# Autodesk Inventor assembly: Assembly_v2
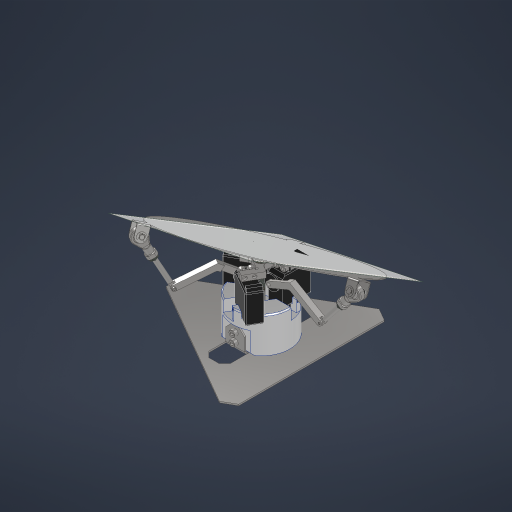
[picture p0: Inventor's stored thumbnail of the model, 512x512]
Saved by Autodesk Inventor 2023 (Build 270158000, 158)
## iProperties
Created: 2023-02-25
Part Number: Assembly_v2
Document SubType Name: Assembly
Designer: roota
Mass: 2527.07 g
Surface Area: 3464.46 cm^2
Volume: 460 cm^3
Density: 5.49363 g/cm^3
Author: roota
## Documents named in this file (20)
- D:\GitHub\NTUST-Mechanical-Design\Ball stabilization mechanism\3D CAD files\Mechanical Part CAD files\Assemblies\Assembly_v2.iam
- D:\GitHub\NTUST-Mechanical-Design\Ball stabilization mechanism\3D CAD files\Mechanical Part CAD files\Static Mechanisms\BalancePlate.ipt
- D:\GitHub\NTUST-Mechanical-Design\Ball stabilization mechanism\3D CAD files\Mechanical Part CAD files\Static Mechanisms\BasePlate.ipt
- D:\GitHub\NTUST-Mechanical-Design\Ball stabilization mechanism\3D CAD files\Mechanical Part CAD files\Static Mechanisms\BaseSupport.ipt
- D:\GitHub\NTUST-Mechanical-Design\Ball stabilization mechanism\3D CAD files\Mechanical Part CAD files\Static Mechanisms\ServoCap.ipt
- D:\GitHub\NTUST-Mechanical-Design\Ball stabilization mechanism\3D CAD files\Electrical Hardware CAD files\SERVO\LDX-335MG_Servo_15kg_cm.ipt
- C:\Users\roota\Documents\Inventor\Content Center Files\R2023\en-US\ISO 10642(1)\ISO 10642 - M8 x  60.ipt
- C:\Users\roota\Documents\Inventor\Content Center Files\R2023\en-US\ISO 4762(2)\ISO 4762 - M5 x 8ISO.ipt
- C:\Users\roota\Documents\Inventor\Content Center Files\R2023\en-US\ISO 4026\ISO 4026 - M3 x 6 - ISO.ipt
- D:\GitHub\NTUST-Mechanical-Design\Ball stabilization mechanism\3D CAD files\Mechanical Part CAD files\Hardware Parts\5mm Bushing.ipt
- D:\GitHub\NTUST-Mechanical-Design\Ball stabilization mechanism\3D CAD files\Mechanical Part CAD files\Hardware Parts\M6x1_THREADED_ROD.ipt
- C:\Users\roota\Documents\Inventor\Content Center Files\R2023\en-US\ISO 4762(2)\ISO 4762 - M2.5 x 8ISO.ipt
- D:\GitHub\NTUST-Mechanical-Design\Ball stabilization mechanism\3D CAD files\Mechanical Part CAD files\Hardware Parts\SELF-LUBRIFICATING ROD END\End_6mm.ipt
- D:\GitHub\NTUST-Mechanical-Design\Ball stabilization mechanism\3D CAD files\Mechanical Part CAD files\Hardware Parts\SELF-LUBRIFICATING ROD END\Ball_6mm.ipt
- D:\GitHub\NTUST-Mechanical-Design\Ball stabilization mechanism\3D CAD files\Mechanical Part CAD files\Static Mechanisms\4mm spacer.ipt
- D:\GitHub\NTUST-Mechanical-Design\Ball stabilization mechanism\3D CAD files\Mechanical Part CAD files\Static Mechanisms\rod pin.ipt
- C:\Users\roota\Documents\Inventor\Content Center Files\R2023\en-US\JIS B 2804 E\_JIS B 2804 E - 5 - 6.ipt
- C:\Users\roota\Documents\Inventor\Content Center Files\R2023\en-US\ISO 4036(2)\ISO 4036 - M6(2).ipt
- D:\GitHub\NTUST-Mechanical-Design\Ball stabilization mechanism\3D CAD files\Mechanical Part CAD files\Hardware Parts\12_1_INCH_TOUCHSCREEN\12inch Touchscreen.ipt
- D:\GitHub\NTUST-Mechanical-Design\Ball stabilization mechanism\3D CAD files\Mechanical Part CAD files\Dynamic Mechanisms\Servo_Strut_v2.ipt
## Components (58 placed, 19 different names)
1. BalancePlate:1 — Mate:19, Mate:20, Mate:21, Mate:22, Mate:23, Mate:24, Mate:26, Mate:28, Mate:30, Mate:31, Flush:1, Flush:2, Mate:44
2. BasePlate:1 — Mate:1, Mate:2, Mate:3, Insert:13, Insert:14, Insert:15, Insert:16, Angle:4, Angle:5
3. BaseSupport:1 — Mate:1, Mate:2, Mate:3, Mate:4, Mate:5, Mate:6, Mate:7, Mate:8, Mate:9, Mate:10, Mate:11, Mate:12, Mate:17, Mate:18, Insert:17, Mate:44
4. ServoCap:1 — Mate:13, Mate:14, Mate:15, Mate:16
5. LDX-335MG_Servo_15kg_cm:1 — Mate:4, Mate:7, Mate:10, Insert:5, Insert:8, Insert:49
6. LDX-335MG_Servo_15kg_cm:2 — Mate:5, Mate:8, Mate:11, Insert:9, Insert:12, Insert:50
7. LDX-335MG_Servo_15kg_cm:3 — Mate:6, Mate:9, Mate:12, Mate:13, Mate:14, Mate:15, Insert:1, Insert:4, Insert:48
8. ISO 10642 M8x60:1 — Mate:16
9. ISO 4762 M5 x 8:1 — Insert:1
10. ISO 4762 M5 x 8:4 — Insert:4
11. ISO 4762 M5 x 8:5 — Insert:5
12. ISO 4762 M5 x 8:8 — Insert:8
13. ISO 4762 M5 x 8:9 — Insert:9
14. ISO 4762 M5 x 8:12 — Insert:12
15. ISO 4762 M5 x 8:13 — Insert:13
16. ISO 4762 M5 x 8:14 — Insert:14
17. ISO 4762 M5 x 8:15 — Insert:15
18. ISO 4762 M5 x 8:16 — Insert:16
19. ISO 4026 M3 x 6:1 — Mate:17
20. ISO 4026 M3 x 6:2 — Mate:18
21. ISO 4026 M3 x 6:3 — Insert:17
22. 5mm Bushing:1 — Insert:27, Mate:36, Mate:38
23. 5mm Bushing:2 — Insert:29, Mate:32, Mate:33, Mate:34
24. 5mm Bushing:3 — Insert:28, Mate:39, Mate:40
25. M6x1_THREADED_ROD:1 — Insert:32, Angle:3, Mate:34, Mate:35
26. M6x1_THREADED_ROD:2 — Insert:31, Angle:2, Mate:36, Mate:43
27. M6x1_THREADED_ROD:3 — Insert:30, Angle:1, Mate:39, Mate:41
28. ISO 4762 M2.5 x 8:1 — Insert:27, Mate:37
29. ISO 4762 M2.5 x 8:2 — Insert:28, Mate:42
30. ISO 4762 M2.5 x 8:3 — Insert:29
31. End_6mm:1 — Insert:30, Tangent:2, Angle:1, Insert:46
32. End_6mm:2 — Insert:31, Tangent:3, Angle:2, Insert:47
33. End_6mm:3 — Insert:32, Tangent:1, Angle:3, Insert:45
34. Ball_6mm:1 — Tangent:1, Insert:34, Insert:35
35. Ball_6mm:2 — Tangent:2, Insert:36, Insert:37
36. Ball_6mm:3 — Tangent:3, Insert:33, Insert:38
37. 4mm spacer:1 — Insert:33
38. 4mm spacer:3 — Insert:34
39. 4mm spacer:4 — Insert:35, Mate:27, Mate:28
40. 4mm spacer:5 — Insert:36
41. 4mm spacer:6 — Insert:37, Mate:29, Mate:30
42. 4mm spacer:7 — Insert:38, Mate:25, Mate:26
43. rod pin:1 — Insert:39, Insert:40, Mate:19, Mate:27
44. rod pin:2 — Insert:41, Insert:42, Mate:20, Mate:25
45. rod pin:3 — Insert:43, Insert:44, Mate:21, Mate:29
46. JIS B 2804 E 5:1 — Insert:39
47. JIS B 2804 E 5:2 — Insert:40, Mate:22
48. JIS B 2804 E 5:3 — Insert:41, Mate:23
49. JIS B 2804 E 5:4 — Insert:42
50. JIS B 2804 E 5:5 — Insert:43, Mate:24
51. JIS B 2804 E 5:6 — Insert:44
52. ISO 4036 M6:1 — Insert:45
53. ISO 4036 M6:2 — Insert:46
54. ISO 4036 M6:3 — Insert:47
55. 12inch Touchscreen:1 — Mate:31, Flush:1, Flush:2, Angle:4, Angle:5
56. Servo_Strut_v2:1 — Insert:48, Mate:37, Mate:38, Mate:43
57. Servo_Strut_v2:2 — Insert:49, Mate:40, Mate:41, Mate:42
58. Servo_Strut_v2:3 — Insert:50, Mate:32, Mate:33, Mate:35
## Relationships (89: Mate 44, Insert 35, Angle 5, Tangent 3, Flush 2)
- Mate:1: BasePlate:1 ↔ BaseSupport:1
- Mate:2: BasePlate:1 ↔ BaseSupport:1
- Mate:3: BasePlate:1 ↔ BaseSupport:1
- Mate:4: BaseSupport:1 ↔ LDX-335MG_Servo_15kg_cm:1
- Mate:5: BaseSupport:1 ↔ LDX-335MG_Servo_15kg_cm:2
- Mate:6: BaseSupport:1 ↔ LDX-335MG_Servo_15kg_cm:3
- Mate:7: BaseSupport:1 ↔ LDX-335MG_Servo_15kg_cm:1
- Mate:8: BaseSupport:1 ↔ LDX-335MG_Servo_15kg_cm:2
- Mate:9: BaseSupport:1 ↔ LDX-335MG_Servo_15kg_cm:3
- Mate:10: BaseSupport:1 ↔ LDX-335MG_Servo_15kg_cm:1
- Mate:11: BaseSupport:1 ↔ LDX-335MG_Servo_15kg_cm:2
- Mate:12: BaseSupport:1 ↔ LDX-335MG_Servo_15kg_cm:3
- Mate:13: ServoCap:1 ↔ LDX-335MG_Servo_15kg_cm:3
- Mate:14: ServoCap:1 ↔ LDX-335MG_Servo_15kg_cm:3
- Mate:15: ServoCap:1 ↔ LDX-335MG_Servo_15kg_cm:3
- Mate:16: ServoCap:1 ↔ ISO 10642 M8x60:1
- Insert:1: LDX-335MG_Servo_15kg_cm:3 ↔ ISO 4762 M5 x 8:1
- Insert:4: LDX-335MG_Servo_15kg_cm:3 ↔ ISO 4762 M5 x 8:4
- Insert:5: LDX-335MG_Servo_15kg_cm:1 ↔ ISO 4762 M5 x 8:5
- Insert:8: LDX-335MG_Servo_15kg_cm:1 ↔ ISO 4762 M5 x 8:8
- Insert:9: LDX-335MG_Servo_15kg_cm:2 ↔ ISO 4762 M5 x 8:9
- Insert:12: LDX-335MG_Servo_15kg_cm:2 ↔ ISO 4762 M5 x 8:12
- Insert:13: BasePlate:1 ↔ ISO 4762 M5 x 8:13
- Insert:14: BasePlate:1 ↔ ISO 4762 M5 x 8:14
- Insert:15: BasePlate:1 ↔ ISO 4762 M5 x 8:15
- Insert:16: BasePlate:1 ↔ ISO 4762 M5 x 8:16
- Mate:17: BaseSupport:1 ↔ ISO 4026 M3 x 6:1
- Mate:18: BaseSupport:1 ↔ ISO 4026 M3 x 6:2
- Insert:17: BaseSupport:1 ↔ ISO 4026 M3 x 6:3
- Insert:27: 5mm Bushing:1 ↔ ISO 4762 M2.5 x 8:1
- Insert:28: 5mm Bushing:3 ↔ ISO 4762 M2.5 x 8:2
- Insert:29: 5mm Bushing:2 ↔ ISO 4762 M2.5 x 8:3
- Insert:30 (-10 mm): M6x1_THREADED_ROD:3 ↔ End_6mm:1
- Insert:31 (-10 mm): M6x1_THREADED_ROD:2 ↔ End_6mm:2
- Insert:32 (-10 mm): M6x1_THREADED_ROD:1 ↔ End_6mm:3
- Tangent:1: End_6mm:3 ↔ Ball_6mm:1
- Tangent:2: End_6mm:1 ↔ Ball_6mm:2
- Tangent:3: End_6mm:2 ↔ Ball_6mm:3
- Insert:33: Ball_6mm:3 ↔ 4mm spacer:1
- Insert:34: Ball_6mm:1 ↔ 4mm spacer:3
- Insert:35: Ball_6mm:1 ↔ 4mm spacer:4
- Insert:36: Ball_6mm:2 ↔ 4mm spacer:5
- Insert:37: Ball_6mm:2 ↔ 4mm spacer:6
- Insert:38: Ball_6mm:3 ↔ 4mm spacer:7
- Insert:39: rod pin:1 ↔ JIS B 2804 E 5:1
- Insert:40: rod pin:1 ↔ JIS B 2804 E 5:2
- Insert:41: rod pin:2 ↔ JIS B 2804 E 5:3
- Insert:42: rod pin:2 ↔ JIS B 2804 E 5:4
- Insert:43: rod pin:3 ↔ JIS B 2804 E 5:5
- Insert:44: rod pin:3 ↔ JIS B 2804 E 5:6
- Mate:19: BalancePlate:1 ↔ rod pin:1
- Mate:20: BalancePlate:1 ↔ rod pin:2
- Mate:21: BalancePlate:1 ↔ rod pin:3
- Mate:22: BalancePlate:1 ↔ JIS B 2804 E 5:2
- Mate:23: BalancePlate:1 ↔ JIS B 2804 E 5:3
- Mate:24: BalancePlate:1 ↔ JIS B 2804 E 5:5
- Mate:25: 4mm spacer:7 ↔ rod pin:2
- Mate:26: BalancePlate:1 ↔ 4mm spacer:7
- Mate:27: 4mm spacer:4 ↔ rod pin:1
- Mate:28: BalancePlate:1 ↔ 4mm spacer:4
- Mate:29: 4mm spacer:6 ↔ rod pin:3
- Mate:30: BalancePlate:1 ↔ 4mm spacer:6
- Angle:1 (0 deg): M6x1_THREADED_ROD:3 ↔ End_6mm:1
- Angle:2 (0 deg): M6x1_THREADED_ROD:2 ↔ End_6mm:2
- Angle:3 (0 deg): M6x1_THREADED_ROD:1 ↔ End_6mm:3
- Insert:45: End_6mm:3 ↔ ISO 4036 M6:1
- Insert:46: End_6mm:1 ↔ ISO 4036 M6:2
- Insert:47: End_6mm:2 ↔ ISO 4036 M6:3
- Mate:31: BalancePlate:1 ↔ 12inch Touchscreen:1
- Flush:1 (-120 mm): BalancePlate:1 ↔ 12inch Touchscreen:1
- Flush:2 (40 mm): BalancePlate:1 ↔ 12inch Touchscreen:1
- Insert:48: LDX-335MG_Servo_15kg_cm:3 ↔ Servo_Strut_v2:1
- Insert:49: LDX-335MG_Servo_15kg_cm:1 ↔ Servo_Strut_v2:2
- Insert:50: LDX-335MG_Servo_15kg_cm:2 ↔ Servo_Strut_v2:3
- Mate:32: 5mm Bushing:2 ↔ Servo_Strut_v2:3
- Mate:33: 5mm Bushing:2 ↔ Servo_Strut_v2:3
- Mate:34: 5mm Bushing:2 ↔ M6x1_THREADED_ROD:1
- Mate:35: M6x1_THREADED_ROD:1 ↔ Servo_Strut_v2:3
- Mate:36: 5mm Bushing:1 ↔ M6x1_THREADED_ROD:2
- Mate:37: ISO 4762 M2.5 x 8:1 ↔ Servo_Strut_v2:1
- Mate:38: 5mm Bushing:1 ↔ Servo_Strut_v2:1
- Mate:39: 5mm Bushing:3 ↔ M6x1_THREADED_ROD:3
- Mate:40: 5mm Bushing:3 ↔ Servo_Strut_v2:2
- Mate:41: M6x1_THREADED_ROD:3 ↔ Servo_Strut_v2:2
- Mate:42: ISO 4762 M2.5 x 8:2 ↔ Servo_Strut_v2:2
- Mate:43: M6x1_THREADED_ROD:2 ↔ Servo_Strut_v2:1
- Angle:4 (120 deg): BasePlate:1 ↔ 12inch Touchscreen:1
- Angle:5 (-100 deg): BasePlate:1 ↔ 12inch Touchscreen:1
- Mate:44 (60 mm): BalancePlate:1 ↔ BaseSupport:1
## Named parameters: AngleX = 30 deg, AngleY = 10 deg
